# Autodesk Inventor assembly: Assembly
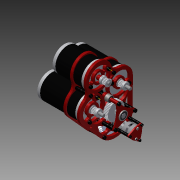
[picture p0: Inventor's stored thumbnail of the model, 180x180]
Saved by Autodesk Inventor 2013 (Build 170138000, 138)
## iProperties
Created: 2013-06-04
Part Number: Assembly
Document SubType Name: Assembly
Designer: mvarma
Author: mvarma
## Documents named in this file (59)
- C:\Users\mvarma\Desktop\GRT 2013-2014 Gearbox\Mark 3\Assembly.iam
- C:\Users\mvarma\Desktop\GRT 2013-2014 Gearbox\Mark 3\Frame Segment.ipt
- C:\Users\mvarma\Desktop\GRT 2013-2014 Gearbox\Mark 3\Plates\Cim Plate.ipt
- C:\Users\mvarma\Desktop\GRT 2013-2014 Gearbox\Mark 3\Wheel Temp.ipt
- C:\Users\mvarma\Desktop\GRT 2013-2014 Gearbox\Mark 3\Motors\Mini CIM Motor.ipt
- C:\Users\mvarma\Desktop\GRT 2013-2014 Gearbox\Mark 3\Motors\CIM Motor.ipt
- C:\Users\mvarma\Desktop\GRT 2013-2014 Gearbox\Mark 3\Pulleys\16T 3mm GT2 - 8mm Key Broach.ipt
- C:\Users\mvarma\Desktop\GRT 2013-2014 Gearbox\Mark 3\Pulleys\48T 3mm GT2 - .375 Hex Broach - Hubless.ipt
- C:\Users\mvarma\Desktop\GRT 2013-2014 Gearbox\Mark 3\Bearings\FR6-2ZZ - Hex.ipt
- C:\Users\mvarma\Desktop\GRT 2013-2014 Gearbox\Mark 3\Spacers\Shim 10 thou .500 Bore.ipt
- C:\Users\mvarma\Desktop\GRT 2013-2014 Gearbox\Mark 3\Bearings\R4-2RS.ipt
- C:\Users\mvarma\Desktop\GRT 2013-2014 Gearbox\Mark 3\Spacers\Belt Shaft Spacer 1.ipt
- C:\Users\mvarma\Desktop\GRT 2013-2014 Gearbox\Mark 3\Plates\Pnuematic Plate.ipt
- C:\Users\mvarma\Desktop\GRT 2013-2014 Gearbox\Mark 3\Spacers\Shim 10 thou .375 Bore.ipt
- C:\Users\mvarma\Desktop\GRT 2013-2014 Gearbox\Mark 3\Bearings\FR6-2RS.ipt
- C:\Users\mvarma\Desktop\GRT 2013-2014 Gearbox\Mark 3\Spacers\Belt Shaft Spacer 2.ipt
- C:\Users\mvarma\Desktop\GRT 2013-2014 Gearbox\Mark 3\Shafts\Cluster Shaft.ipt
- C:\Users\mvarma\Desktop\GRT 2013-2014 Gearbox\Mark 3\Gears\15T 20DP - .375 Hex Bore.ipt
- C:\Users\mvarma\Desktop\GRT 2013-2014 Gearbox\Mark 3\Gears\28T 20DP - .375 Hex Bore.ipt
- C:\Users\mvarma\Desktop\GRT 2013-2014 Gearbox\Mark 3\Spacers\MiniCim Spacer.ipt
- C:\Users\mvarma\Desktop\GRT 2013-2014 Gearbox\Mark 3\Spacers\Cim Spacer.ipt
- C:\Users\mvarma\Desktop\GRT 2013-2014 Gearbox\Mark 3\Plates\Mounting Plate.ipt
- C:\Users\mvarma\Desktop\GRT 2013-2014 Gearbox\Mark 3\Gears\35T 20DP - .188 Ball Shifting Bore.ipt
- C:\Users\mvarma\Desktop\GRT 2013-2014 Gearbox\Mark 3\Gears\48T 20DP - .188 Ball Shifting Bore.ipt
- C:\Users\mvarma\Desktop\GRT 2013-2014 Gearbox\Mark 3\Bearings\Thrust Bearing Washer - .6250 Bore.ipt
- C:\Users\mvarma\Desktop\GRT 2013-2014 Gearbox\Mark 3\Bearings\R10-Open.ipt
- C:\Users\mvarma\Desktop\GRT 2013-2014 Gearbox\Mark 3\Shafts\Output Shaft.ipt
- C:\Users\mvarma\Desktop\GRT 2013-2014 Gearbox\Mark 3\Pneumatic\Pneumatic Connector -Actuator Side.ipt
- C:\Users\mvarma\Desktop\GRT 2013-2014 Gearbox\Mark 3\Pneumatic\Mouning Standoff.ipt
- C:\Users\mvarma\Desktop\GRT 2013-2014 Gearbox\Mark 3\Bearings\FR8-2RS.ipt
- C:\Users\mvarma\Desktop\GRT 2013-2014 Gearbox\Mark 3\Spacers\Shim 10 thou .625 Bore.ipt
- C:\Users\mvarma\Desktop\GRT 2013-2014 Gearbox\Mark 3\Shafts\Output Shaft Insert.ipt
- C:\Users\mvarma\Desktop\GRT 2013-2014 Gearbox\Mark 3\Shafts\Ball Shifting Shaft.ipt
- C:\Users\mvarma\Desktop\GRT 2013-2014 Gearbox\Mark 3\Pneumatic\Pneumatic Connector -Shaft Side Cover.ipt
- C:\Users\mvarma\Desktop\GRT 2013-2014 Gearbox\Mark 3\Bolts\Button Head Cap Screw 4-40 Thread .125 Length.ipt
- C:\Users\mvarma\Desktop\GRT 2013-2014 Gearbox\Mark 3\Encoder\S4-120-250-N-S-B.ipt
- C:\Users\mvarma\Desktop\GRT 2013-2014 Gearbox\Mark 3\Shafts\Flexible Shaft Coupler 6208K411.ipt
- C:\Users\mvarma\Desktop\GRT 2013-2014 Gearbox\Mark 3\Encoder\Encoder Mount.ipt
- C:\Users\mvarma\Desktop\GRT 2013-2014 Gearbox\Mark 3\Bolts\Socket Head Cap Screw 6-32 Thread 1.500 Length.ipt
- C:\Users\mvarma\Desktop\GRT 2013-2014 Gearbox\Mark 3\Bearings\R3-2RS.ipt
- C:\Users\mvarma\Desktop\GRT 2013-2014 Gearbox\Mark 3\.0625 Spring Pin .2500 Long.ipt
- C:\Users\mvarma\Desktop\GRT 2013-2014 Gearbox\Mark 3\Pneumatic\FO_020_318_4F_2_03.iam
- C:\Users\mvarma\Desktop\GRT 2013-2014 Gearbox\Mark 3\Pneumatic\Mounting Plate.ipt
- C:\Users\mvarma\Desktop\GRT 2013-2014 Gearbox\Mark 3\Pem Nuts\4-40 Clinch Style Pem Nut .091 Minimum Panel Thickness.ipt
- C:\Users\mvarma\Desktop\GRT 2013-2014 Gearbox\Mark 3\Bolts\Socket Head Cap Screw 4-40 Thread 1.000 Length.ipt
- C:\Users\mvarma\Desktop\GRT 2013-2014 Gearbox\Mark 3\Bolts\Socket Head Cap Screw 6-32 Thread 2.250 Length.ipt
- C:\Users\mvarma\Desktop\GRT 2013-2014 Gearbox\Mark 3\Bolts\Socket Head Cap Screw 10-32 Thread .500 Length.ipt
- C:\Users\mvarma\Desktop\GRT 2013-2014 Gearbox\Mark 3\Spacers\Cluster Shaft Spacer.ipt
- C:\Users\mvarma\Desktop\GRT 2013-2014 Gearbox\Mark 3\Shafts\Tensioning Shaft.ipt
- C:\Users\mvarma\Desktop\GRT 2013-2014 Gearbox\Base Parts\Pulleys\22T 5mm GT2 - .500 Hex Broach.ipt
- C:\Users\mvarma\Desktop\GRT 2013-2014 Gearbox\Mark 3\Shafts\Output Shaft Hex Sleave.ipt
- C:\Users\mvarma\Desktop\GRT 2013-2014 Gearbox\Base Parts\Shafts\Base OutputShaft.ipt
- C:\Users\mvarma\Desktop\GRT 2013-2014 Gearbox\Mark 3\Bolts\Button Head Cap Screw .25-20 Thread 3.500 Length.ipt
- C:\Users\mvarma\Desktop\GRT 2013-2014 Gearbox\Mark 3\Spacers\Washer 50 thou .250 Bore.ipt
- C:\Users\mvarma\Desktop\GRT 2013-2014 Gearbox\Mark 3\Plates\Supporting Plate Standoff.ipt
- C:\Users\mvarma\Desktop\GRT 2013-2014 Gearbox\Mark 3\Plates\Main Connecting Standoff.ipt
- C:\Users\mvarma\Desktop\GRT 2013-2014 Gearbox\Mark 3\Pem Nuts\10-32 Clinch Style Pem Nut .091 Minimum Panel Thickness.ipt
- C:\Users\mvarma\Desktop\GRT 2013-2014 Gearbox\Mark 3\Bolts\Socket Head Cap Screw 10-32 Thread 3.000 Length.ipt
- C:\Users\mvarma\Desktop\GRT 2013-2014 Gearbox\Mark 3\Bolts\Socket Head Cap Screw 10-32 Thread 1.750 Length.ipt
## Components (100 placed, 57 different names)
1. Frame Segment:1 — Mate:1, Mate:2, Mate:70, Mate:71, Mate:339, Mate:340, Mate:342, Mate:343, Mate:344, Angle:6
2. Wheel Temp:1 — Mate:2, Mate:346, Mate:349
3. 22T 5mm GT2 - .500 Hex Broach:1 — Mate:339, Mate:340
4. FR8-2RS:3 — Mate:342, Mate:343, Mate:346, Mate:347
5. Output Shaft Hex Sleave:1 — Mate:344, Mate:345, Flush:26, Flush:27
6. Base OutputShaft:1 — Mate:347, Mate:348, Flush:27, Mate:349, Mate:350, Mate:352
7. Button Head Cap Screw .25-20 Thread 3.500 Length:1 — Mate:350, Mate:351, Mate:353
8. Washer 50 thou .250 Bore:1 — Mate:351, Mate:352, Mate:353
9. Supporting Plate Standoff:1 — Mate:360, Mate:361
10. Supporting Plate Standoff:2 — Mate:358, Mate:359
11. Tensioning Shaft:1 — Mate:362, Mate:363, Mate:364, Mate:365, Mate:366, Mate:367
12. Main Connecting Standoff:1 — Mate:370, Mate:371
13. Main Connecting Standoff:2 — Mate:372, Mate:373
14. Main Connecting Standoff:3 — Mate:368, Mate:369
15. 10-32 Clinch Style Pem Nut .091 Minimum Panel Thickness:1 — Mate:378, Mate:379
16. 10-32 Clinch Style Pem Nut .091 Minimum Panel Thickness:2 — Mate:376, Mate:377
17. 10-32 Clinch Style Pem Nut .091 Minimum Panel Thickness:3 — Mate:374, Mate:375
18. Socket Head Cap Screw 10-32 Thread 3.000 Length:1 — Mate:384, Mate:385
19. Socket Head Cap Screw 10-32 Thread 3.000 Length:2 — Mate:382, Mate:383
20. Socket Head Cap Screw 10-32 Thread 3.000 Length:3 — Mate:380, Mate:381
21. 10-32 Clinch Style Pem Nut .091 Minimum Panel Thickness:4 — Mate:387, Mate:388
22. 10-32 Clinch Style Pem Nut .091 Minimum Panel Thickness:5 — Mate:386, Mate:389
23. Socket Head Cap Screw 10-32 Thread 1.750 Length:1 — Mate:391, Mate:392, Mate:394
24. Socket Head Cap Screw 10-32 Thread 1.750 Length:2 — Mate:390, Mate:393, Mate:396
25. Main Connecting Standoff:4 — Mate:396, Mate:397
26. Main Connecting Standoff:5 — Mate:394, Mate:395
27. Main Connecting Standoff:6 — Mate:398, Mate:401
28. Main Connecting Standoff:7 — Mate:402, Mate:403
29. 10-32 Clinch Style Pem Nut .091 Minimum Panel Thickness:6 — Mate:404, Mate:407
30. 10-32 Clinch Style Pem Nut .091 Minimum Panel Thickness:7 — Mate:405, Mate:406
31. Socket Head Cap Screw 10-32 Thread 1.750 Length:3 — Mate:410, Mate:411
32. Socket Head Cap Screw 10-32 Thread 1.750 Length:4 — Mate:408, Mate:409
33. R10-Open:2 — Mate:218, Mate:219
34. R10-Open:1 — Mate:217, Mate:220, Mate:224
35. FR8-2RS:1 — Mate:203, Mate:204, Mate:205, Mate:208
36. FR8-2RS:2 — Mate:215, Mate:216, Mate:229, Mate:275
37. FR6-2RS:2 — Mate:74, Mate:75, Flush:24, Mate:328
38. FR6-2RS:1 — Mate:36, Mate:37, Mate:38
39. FR6-2ZZ - Hex:1 — Mate:19, Mate:20, Mate:22, Mate:44, Mate:324, Mate:325, Mate:327
40. R4-2RS:1 — Mate:27, Mate:28, Flush:9
41. R4-2RS:2 — Mate:27, Mate:28, Mate:42, Mate:364
42. Socket Head Cap Screw 6-32 Thread 1.500 Length:1 — Mate:268, Mate:270
43. Socket Head Cap Screw 6-32 Thread 1.500 Length:2 — Mate:269, Mate:271
44. S4-120-250-N-S-B:1 — Mate:263, Mate:267, Mate:272, Mate:273
45. Flexible Shaft Coupler 6208K411:1 — Mate:264, Mate:265, Mate:267
46. Encoder Mount:1 — Mate:268, Mate:269, Mate:270, Mate:271, Mate:272, Mate:273, Mate:274
47. Mounting Plate:1 — Mate:70, Mate:71, Mate:74, Mate:75, Mate:177, Mate:203, Mate:204, Mate:274, Mate:368, Mate:369, Mate:370, Mate:371, Mate:374, Mate:375, Mate:376, Mate:377, Mate:378, Mate:379, Mate:386, Mate:387, Mate:388, Mate:389, Mate:395, Mate:397, Mate:401, Mate:402, Mate:403, Mate:404, Mate:405, Mate:406, Mate:407
48. Pnuematic Plate:1 — Mate:32, Mate:34, Mate:36, Mate:37, Mate:43, Mate:367, Mate:380, Mate:381, Mate:382, Mate:383, Mate:384, Mate:385
49. Cim Plate:1 — Mate:1, Mate:3, Mate:4, Mate:5, Mate:6, Mate:7, Mate:8, Mate:9, Mate:10, Mate:11, Mate:15, Mate:19, Mate:20, Mate:21, Mate:31, Mate:32, Mate:46, Mate:215, Mate:216, Mate:288, Mate:289, Mate:292, Mate:293, Mate:294, Mate:295, Mate:312, Mate:313, Mate:314, Mate:315, Mate:316, Mate:317, Mate:318, Mate:319, Mate:320, Mate:321, Mate:322, Mate:323, Mate:358, Mate:359, Mate:360, Mate:361, Mate:362, Mate:363, Mate:372, Mate:373, Mate:390, Mate:391, Mate:392, Mate:393, Mate:398, Angle:6, Mate:408, Mate:409, Mate:410, Mate:411
50. 16T 3mm GT2 - 8mm Key Broach:1 — Mate:13, Flush:5, Flush:6
51. 16T 3mm GT2 - 8mm Key Broach:2 — Mate:12, Flush:4, Flush:7
52. 16T 3mm GT2 - 8mm Key Broach:3 — Mate:14, Flush:3, Mate:311
53. 48T 3mm GT2 - .375 Hex Broach - Hubless:1 — Mate:15, Flush:6, Flush:7, Mate:23, Flush:9, Mate:310, Mate:311, Mate:329
54. Socket Head Cap Screw 10-32 Thread .500 Length:1 — Mate:316, Mate:317
55. Socket Head Cap Screw 10-32 Thread .500 Length:2 — Mate:320, Mate:321
56. Socket Head Cap Screw 10-32 Thread .500 Length:3 — Mate:322, Mate:323
57. Socket Head Cap Screw 10-32 Thread .500 Length:4 — Mate:318, Mate:319
58. Socket Head Cap Screw 10-32 Thread .500 Length:5 — Mate:312, Mate:313
59. Socket Head Cap Screw 10-32 Thread .500 Length:6 — Mate:314, Mate:315
60. Mini CIM Motor:1 — Mate:3, Mate:4, Mate:5, Mate:14, Flush:3, Mate:51, Mate:52
61. CIM Motor:1 — Mate:9, Mate:10, Mate:11, Mate:12, Flush:4, Mate:53, Mate:54, Mate:177
62. CIM Motor:2 — Mate:6, Mate:7, Mate:8, Mate:13, Flush:5, Mate:55, Mate:56
63. Cluster Shaft Spacer:1 — Mate:327, Mate:328
64. Thrust Bearing Washer - .6250 Bore:3 — Mate:222, Mate:223, Mate:224
65. Thrust Bearing Washer - .6250 Bore:4 — Mate:225, Mate:226, Mate:228
66. Belt Shaft Spacer 1:1 — Mate:31, Mate:365
67. Belt Shaft Spacer 2:1 — Mate:42, Mate:366
68. MiniCim Spacer:1 — Mate:51, Mate:52
69. Cim Spacer:1 — Mate:53, Mate:54
70. Cim Spacer:2 — Mate:55, Mate:56
71. Shim 10 thou .500 Bore:2 — Mate:207, Mate:208, Mate:341
72. Shim 10 thou .625 Bore:2 — Mate:227, Mate:228, Mate:275
73. Shim 10 thou .375 Bore:1 — Mate:34, Mate:38, Mate:329
74. Shim 10 thou .500 Bore:1 — Mate:21, Mate:22, Mate:23
75. Output Shaft:2 — Mate:205, Mate:207, Mate:213, Mate:214, Mate:223, Mate:225, Mate:227, Mate:229, Mate:230, Mate:231, Mate:341, Mate:345, Flush:26, Mate:348
76. Cluster Shaft:1 — Mate:43, Mate:44, Angle:4, Mate:263, Mate:264, Mate:265, Mate:310, Flush:24
77. Output Shaft Insert:1 — Mate:230, Mate:231, Mate:232, Flush:23
78. Ball Shifting Shaft:1 — Mate:232, Mate:248, Flush:23, Mate:276, Mate:278, Mate:279, Mate:281
79. 35T 20DP - .188 Ball Shifting Bore:1 — Mate:213, Mate:218, Mate:219, Mate:222
80. 48T 20DP - .188 Ball Shifting Bore:1 — Mate:214, Mate:217, Mate:220, Mate:226
81. 15T 20DP - .375 Hex Bore:1 — Angle:4, Angle:5, Mate:324, Mate:325, Mate:326
82. 28T 20DP - .375 Hex Bore:1 — Mate:46, Angle:5, Mate:326
83. FO_020_318_4F_2_03:1 [sub-assembly] — Mate:282, Mate:283, Mate:284, Mate:286, Mate:287, Mate:302, Mate:303
84. 4-40 Clinch Style Pem Nut .091 Minimum Panel Thickness:1 — Mate:297, Mate:298, Mate:300
85. 4-40 Clinch Style Pem Nut .091 Minimum Panel Thickness:2 — Mate:296, Mate:299, Mate:301
86. Socket Head Cap Screw 4-40 Thread 1.000 Length:1 — Mate:301, Mate:303
87. Socket Head Cap Screw 4-40 Thread 1.000 Length:2 — Mate:300, Mate:302
88. Socket Head Cap Screw 6-32 Thread 2.250 Length:1 — Mate:304, Mate:308, Mate:338
89. Socket Head Cap Screw 6-32 Thread 2.250 Length:2 — Mate:307, Mate:400
90. Socket Head Cap Screw 6-32 Thread 2.250 Length:3 — Mate:309, Mate:399
91. Mounting Plate:2 — Mate:286, Mate:287, Mate:291, Mate:296, Mate:297, Mate:298, Mate:299, Mate:304, Mate:307, Mate:308, Mate:309
92. Mouning Standoff:1 — Mate:288, Mate:289, Mate:291, Mate:399
93. Mouning Standoff:2 — Mate:294, Mate:295, Mate:338
94. Mouning Standoff:3 — Mate:292, Mate:293, Mate:400
95. .0625 Spring Pin .2500 Long:1 — Mate:278, Mate:279
96. R3-2RS:1 — Mate:276, Mate:280, Mate:281
97. Button Head Cap Screw 4-40 Thread .125 Length:1 — Mate:259, Mate:260
98. Button Head Cap Screw 4-40 Thread .125 Length:2 — Mate:261, Mate:262
99. Pneumatic Connector -Actuator Side:1 — Mate:249, Mate:250, Mate:258, Mate:259, Mate:280, Mate:282, Mate:283, Mate:284
100. Pneumatic Connector -Shaft Side Cover:1 — Mate:248, Mate:249, Mate:250, Mate:258, Mate:260, Mate:261, Mate:262
## Relationships (219: Mate 206, Flush 10, Angle 3)
- Mate:1: Frame Segment:1 ↔ Cim Plate:1
- Mate:2: Frame Segment:1 ↔ Wheel Temp:1
- Mate:3: Cim Plate:1 ↔ Mini CIM Motor:1
- Mate:4: Cim Plate:1 ↔ Mini CIM Motor:1
- Mate:5: Cim Plate:1 ↔ Mini CIM Motor:1
- Mate:6: Cim Plate:1 ↔ CIM Motor:2
- Mate:7: Cim Plate:1 ↔ CIM Motor:2
- Mate:8: Cim Plate:1 ↔ CIM Motor:2
- Mate:9: Cim Plate:1 ↔ CIM Motor:1
- Mate:10: Cim Plate:1 ↔ CIM Motor:1
- Mate:11: Cim Plate:1 ↔ CIM Motor:1
- Mate:12: 16T 3mm GT2 - 8mm Key Broach:2 ↔ CIM Motor:1
- Mate:13: 16T 3mm GT2 - 8mm Key Broach:1 ↔ CIM Motor:2
- Mate:14: 16T 3mm GT2 - 8mm Key Broach:3 ↔ Mini CIM Motor:1
- Flush:3: 16T 3mm GT2 - 8mm Key Broach:3 ↔ Mini CIM Motor:1
- Flush:4: 16T 3mm GT2 - 8mm Key Broach:2 ↔ CIM Motor:1
- Flush:5: 16T 3mm GT2 - 8mm Key Broach:1 ↔ CIM Motor:2
- Mate:15: Cim Plate:1 ↔ 48T 3mm GT2 - .375 Hex Broach - Hubless:1
- Flush:6: 16T 3mm GT2 - 8mm Key Broach:1 ↔ 48T 3mm GT2 - .375 Hex Broach - Hubless:1
- Flush:7: 16T 3mm GT2 - 8mm Key Broach:2 ↔ 48T 3mm GT2 - .375 Hex Broach - Hubless:1
- Mate:19: FR6-2ZZ - Hex:1 ↔ Cim Plate:1
- Mate:20: FR6-2ZZ - Hex:1 ↔ Cim Plate:1
- Mate:21: Cim Plate:1 ↔ Shim 10 thou .500 Bore:1
- Mate:22: FR6-2ZZ - Hex:1 ↔ Shim 10 thou .500 Bore:1
- Mate:23: 48T 3mm GT2 - .375 Hex Broach - Hubless:1 ↔ Shim 10 thou .500 Bore:1
- Mate:27: R4-2RS:1 ↔ R4-2RS:2
- Mate:28: R4-2RS:1 ↔ R4-2RS:2
- Flush:9: R4-2RS:1 ↔ 48T 3mm GT2 - .375 Hex Broach - Hubless:1
- Mate:31: Cim Plate:1 ↔ Belt Shaft Spacer 1:1
- Mate:32: Pnuematic Plate:1 ↔ Cim Plate:1
- Mate:34: Pnuematic Plate:1 ↔ Shim 10 thou .375 Bore:1
- Mate:36: FR6-2RS:1 ↔ Pnuematic Plate:1
- Mate:37: FR6-2RS:1 ↔ Pnuematic Plate:1
- Mate:38: FR6-2RS:1 ↔ Shim 10 thou .375 Bore:1
- Mate:42: R4-2RS:2 ↔ Belt Shaft Spacer 2:1
- Mate:43: Pnuematic Plate:1 ↔ Cluster Shaft:1
- Mate:44: FR6-2ZZ - Hex:1 ↔ Cluster Shaft:1
- Mate:46: Cim Plate:1 ↔ 28T 20DP - .375 Hex Bore:1
- Angle:4 (0 deg): Cluster Shaft:1 ↔ 15T 20DP - .375 Hex Bore:1
- Angle:5 (0 deg): 15T 20DP - .375 Hex Bore:1 ↔ 28T 20DP - .375 Hex Bore:1
- Mate:51: Mini CIM Motor:1 ↔ MiniCim Spacer:1
- Mate:52: Mini CIM Motor:1 ↔ MiniCim Spacer:1
- Mate:53: CIM Motor:1 ↔ Cim Spacer:1
- Mate:54: CIM Motor:1 ↔ Cim Spacer:1
- Mate:55: CIM Motor:2 ↔ Cim Spacer:2
- Mate:56: CIM Motor:2 ↔ Cim Spacer:2
- Mate:70: Frame Segment:1 ↔ Mounting Plate:1
- Mate:71: Frame Segment:1 ↔ Mounting Plate:1
- Mate:74: FR6-2RS:2 ↔ Mounting Plate:1
- Mate:75: FR6-2RS:2 ↔ Mounting Plate:1
- Mate:177: Mounting Plate:1 ↔ CIM Motor:1
- Mate:203: FR8-2RS:1 ↔ Mounting Plate:1
- Mate:204: FR8-2RS:1 ↔ Mounting Plate:1
- Mate:205: FR8-2RS:1 ↔ Output Shaft:2
- Mate:207: Shim 10 thou .500 Bore:2 ↔ Output Shaft:2
- Mate:208: FR8-2RS:1 ↔ Shim 10 thou .500 Bore:2
- Mate:213: Output Shaft:2 ↔ 35T 20DP - .188 Ball Shifting Bore:1
- Mate:214: Output Shaft:2 ↔ 48T 20DP - .188 Ball Shifting Bore:1
- Mate:215: FR8-2RS:2 ↔ Cim Plate:1
- Mate:216: FR8-2RS:2 ↔ Cim Plate:1
- Mate:217: R10-Open:1 ↔ 48T 20DP - .188 Ball Shifting Bore:1
- Mate:218: R10-Open:2 ↔ 35T 20DP - .188 Ball Shifting Bore:1
- Mate:219: R10-Open:2 ↔ 35T 20DP - .188 Ball Shifting Bore:1
- Mate:220: R10-Open:1 ↔ 48T 20DP - .188 Ball Shifting Bore:1
- Mate:222: Thrust Bearing Washer - .6250 Bore:3 ↔ 35T 20DP - .188 Ball Shifting Bore:1
- Mate:223: Thrust Bearing Washer - .6250 Bore:3 ↔ Output Shaft:2
- Mate:224: R10-Open:1 ↔ Thrust Bearing Washer - .6250 Bore:3
- Mate:225: Thrust Bearing Washer - .6250 Bore:4 ↔ Output Shaft:2
- Mate:226: Thrust Bearing Washer - .6250 Bore:4 ↔ 48T 20DP - .188 Ball Shifting Bore:1
- Mate:227: Shim 10 thou .625 Bore:2 ↔ Output Shaft:2
- Mate:228: Thrust Bearing Washer - .6250 Bore:4 ↔ Shim 10 thou .625 Bore:2
- Mate:229: FR8-2RS:2 ↔ Output Shaft:2
- Mate:230: Output Shaft:2 ↔ Output Shaft Insert:1
- Mate:231: Output Shaft:2 ↔ Output Shaft Insert:1
- Mate:232: Output Shaft Insert:1 ↔ Ball Shifting Shaft:1
- Mate:248: Ball Shifting Shaft:1 ↔ Pneumatic Connector -Shaft Side Cover:1
- Mate:249: Pneumatic Connector -Actuator Side:1 ↔ Pneumatic Connector -Shaft Side Cover:1
- Mate:250: Pneumatic Connector -Actuator Side:1 ↔ Pneumatic Connector -Shaft Side Cover:1
- Flush:23: Output Shaft Insert:1 ↔ Ball Shifting Shaft:1
- Mate:258: Pneumatic Connector -Actuator Side:1 ↔ Pneumatic Connector -Shaft Side Cover:1
- Mate:259: Button Head Cap Screw 4-40 Thread .125 Length:1 ↔ Pneumatic Connector -Actuator Side:1
- Mate:260: Button Head Cap Screw 4-40 Thread .125 Length:1 ↔ Pneumatic Connector -Shaft Side Cover:1
- Mate:261: Button Head Cap Screw 4-40 Thread .125 Length:2 ↔ Pneumatic Connector -Shaft Side Cover:1
- Mate:262: Button Head Cap Screw 4-40 Thread .125 Length:2 ↔ Pneumatic Connector -Shaft Side Cover:1
- Mate:263: S4-120-250-N-S-B:1 ↔ Cluster Shaft:1
- Mate:264: Flexible Shaft Coupler 6208K411:1 ↔ Cluster Shaft:1
- Mate:265: Flexible Shaft Coupler 6208K411:1 ↔ Cluster Shaft:1
- Mate:267: S4-120-250-N-S-B:1 ↔ Flexible Shaft Coupler 6208K411:1
- Mate:268: Socket Head Cap Screw 6-32 Thread 1.500 Length:1 ↔ Encoder Mount:1
- Mate:269: Socket Head Cap Screw 6-32 Thread 1.500 Length:2 ↔ Encoder Mount:1
- Mate:270: Socket Head Cap Screw 6-32 Thread 1.500 Length:1 ↔ Encoder Mount:1
- Mate:271: Socket Head Cap Screw 6-32 Thread 1.500 Length:2 ↔ Encoder Mount:1
- Mate:272: S4-120-250-N-S-B:1 ↔ Encoder Mount:1
- Mate:273: S4-120-250-N-S-B:1 ↔ Encoder Mount:1
- Mate:274: Encoder Mount:1 ↔ Mounting Plate:1
- Mate:275: FR8-2RS:2 ↔ Shim 10 thou .625 Bore:2
- Mate:276: Ball Shifting Shaft:1 ↔ R3-2RS:1
- Mate:278: Ball Shifting Shaft:1 ↔ .0625 Spring Pin .2500 Long:1
- Mate:279: Ball Shifting Shaft:1 ↔ .0625 Spring Pin .2500 Long:1
- Mate:280: R3-2RS:1 ↔ Pneumatic Connector -Actuator Side:1
- Mate:281: Ball Shifting Shaft:1 ↔ R3-2RS:1
- Mate:282: FO_020_318_4F_2_03:1 ↔ Pneumatic Connector -Actuator Side:1
- Mate:283: FO_020_318_4F_2_03:1 ↔ Pneumatic Connector -Actuator Side:1
- Mate:284: FO_020_318_4F_2_03:1 ↔ Pneumatic Connector -Actuator Side:1
- Mate:286: FO_020_318_4F_2_03:1 ↔ Mounting Plate:2
- Mate:287: FO_020_318_4F_2_03:1 ↔ Mounting Plate:2
- Mate:288: Cim Plate:1 ↔ Mouning Standoff:1
- Mate:289: Cim Plate:1 ↔ Mouning Standoff:1
- Mate:291: Mounting Plate:2 ↔ Mouning Standoff:1
- Mate:292: Cim Plate:1 ↔ Mouning Standoff:3
- Mate:293: Cim Plate:1 ↔ Mouning Standoff:3
- Mate:294: Cim Plate:1 ↔ Mouning Standoff:2
- Mate:295: Cim Plate:1 ↔ Mouning Standoff:2
- Mate:296: 4-40 Clinch Style Pem Nut .091 Minimum Panel Thickness:2 ↔ Mounting Plate:2
- Mate:297: 4-40 Clinch Style Pem Nut .091 Minimum Panel Thickness:1 ↔ Mounting Plate:2
- Mate:298: 4-40 Clinch Style Pem Nut .091 Minimum Panel Thickness:1 ↔ Mounting Plate:2
- Mate:299: 4-40 Clinch Style Pem Nut .091 Minimum Panel Thickness:2 ↔ Mounting Plate:2
- Mate:300: 4-40 Clinch Style Pem Nut .091 Minimum Panel Thickness:1 ↔ Socket Head Cap Screw 4-40 Thread 1.000 Length:2
- Mate:301: 4-40 Clinch Style Pem Nut .091 Minimum Panel Thickness:2 ↔ Socket Head Cap Screw 4-40 Thread 1.000 Length:1
- Mate:302: FO_020_318_4F_2_03:1 ↔ Socket Head Cap Screw 4-40 Thread 1.000 Length:2
- Mate:303: FO_020_318_4F_2_03:1 ↔ Socket Head Cap Screw 4-40 Thread 1.000 Length:1
- Mate:304: Socket Head Cap Screw 6-32 Thread 2.250 Length:1 ↔ Mounting Plate:2
- Mate:307: Socket Head Cap Screw 6-32 Thread 2.250 Length:2 ↔ Mounting Plate:2
- Mate:308: Socket Head Cap Screw 6-32 Thread 2.250 Length:1 ↔ Mounting Plate:2
- Mate:309: Socket Head Cap Screw 6-32 Thread 2.250 Length:3 ↔ Mounting Plate:2
- Mate:310: 48T 3mm GT2 - .375 Hex Broach - Hubless:1 ↔ Cluster Shaft:1
- Mate:311: 16T 3mm GT2 - 8mm Key Broach:3 ↔ 48T 3mm GT2 - .375 Hex Broach - Hubless:1
- Mate:312: Cim Plate:1 ↔ Socket Head Cap Screw 10-32 Thread .500 Length:5
- Mate:313: Cim Plate:1 ↔ Socket Head Cap Screw 10-32 Thread .500 Length:5
- Mate:314: Cim Plate:1 ↔ Socket Head Cap Screw 10-32 Thread .500 Length:6
- Mate:315: Cim Plate:1 ↔ Socket Head Cap Screw 10-32 Thread .500 Length:6
- Mate:316: Cim Plate:1 ↔ Socket Head Cap Screw 10-32 Thread .500 Length:1
- Mate:317: Cim Plate:1 ↔ Socket Head Cap Screw 10-32 Thread .500 Length:1
- Mate:318: Cim Plate:1 ↔ Socket Head Cap Screw 10-32 Thread .500 Length:4
- Mate:319: Cim Plate:1 ↔ Socket Head Cap Screw 10-32 Thread .500 Length:4
- Mate:320: Cim Plate:1 ↔ Socket Head Cap Screw 10-32 Thread .500 Length:2
- Mate:321: Cim Plate:1 ↔ Socket Head Cap Screw 10-32 Thread .500 Length:2
- Mate:322: Cim Plate:1 ↔ Socket Head Cap Screw 10-32 Thread .500 Length:3
- Mate:323: Cim Plate:1 ↔ Socket Head Cap Screw 10-32 Thread .500 Length:3
- Mate:324: FR6-2ZZ - Hex:1 ↔ 15T 20DP - .375 Hex Bore:1
- Mate:325: FR6-2ZZ - Hex:1 ↔ 15T 20DP - .375 Hex Bore:1
- Mate:326: 15T 20DP - .375 Hex Bore:1 ↔ 28T 20DP - .375 Hex Bore:1
- Mate:327: FR6-2ZZ - Hex:1 ↔ Cluster Shaft Spacer:1
- Flush:24: FR6-2RS:2 ↔ Cluster Shaft:1
- Mate:328: FR6-2RS:2 ↔ Cluster Shaft Spacer:1
- Mate:329: 48T 3mm GT2 - .375 Hex Broach - Hubless:1 ↔ Shim 10 thou .375 Bore:1
- Mate:338: Socket Head Cap Screw 6-32 Thread 2.250 Length:1 ↔ Mouning Standoff:2
- Mate:339: Frame Segment:1 ↔ 22T 5mm GT2 - .500 Hex Broach:1
- Mate:340: Frame Segment:1 ↔ 22T 5mm GT2 - .500 Hex Broach:1
- Mate:341: Shim 10 thou .500 Bore:2 ↔ Output Shaft:2
- Mate:342: Frame Segment:1 ↔ FR8-2RS:3
- Mate:343: Frame Segment:1 ↔ FR8-2RS:3
- Mate:344: Frame Segment:1 ↔ Output Shaft Hex Sleave:1
- Mate:345: Output Shaft Hex Sleave:1 ↔ Output Shaft:2
- Flush:26: Output Shaft Hex Sleave:1 ↔ Output Shaft:2
- Mate:346: Wheel Temp:1 ↔ FR8-2RS:3
- Mate:347: FR8-2RS:3 ↔ Base OutputShaft:1
- Mate:348: Base OutputShaft:1 ↔ Output Shaft:2
- Flush:27: Output Shaft Hex Sleave:1 ↔ Base OutputShaft:1
- Mate:349: Wheel Temp:1 ↔ Base OutputShaft:1
- Mate:350: Base OutputShaft:1 ↔ Button Head Cap Screw .25-20 Thread 3.500 Length:1
- Mate:351: Button Head Cap Screw .25-20 Thread 3.500 Length:1 ↔ Washer 50 thou .250 Bore:1
- Mate:352: Base OutputShaft:1 ↔ Washer 50 thou .250 Bore:1
- Mate:353: Button Head Cap Screw .25-20 Thread 3.500 Length:1 ↔ Washer 50 thou .250 Bore:1
- Mate:358: Supporting Plate Standoff:2 ↔ Cim Plate:1
- Mate:359: Supporting Plate Standoff:2 ↔ Cim Plate:1
- Mate:360: Supporting Plate Standoff:1 ↔ Cim Plate:1
- Mate:361: Supporting Plate Standoff:1 ↔ Cim Plate:1
- Mate:362: Tensioning Shaft:1 ↔ Cim Plate:1
- Mate:363: Tensioning Shaft:1 ↔ Cim Plate:1
- Mate:364: Tensioning Shaft:1 ↔ R4-2RS:2
- Mate:365: Tensioning Shaft:1 ↔ Belt Shaft Spacer 1:1
- Mate:366: Tensioning Shaft:1 ↔ Belt Shaft Spacer 2:1
- Mate:367: Tensioning Shaft:1 ↔ Pnuematic Plate:1
- Mate:368: Main Connecting Standoff:3 ↔ Mounting Plate:1
- Mate:369: Main Connecting Standoff:3 ↔ Mounting Plate:1
- Mate:370: Main Connecting Standoff:1 ↔ Mounting Plate:1
- Mate:371: Main Connecting Standoff:1 ↔ Mounting Plate:1
- Mate:372: Main Connecting Standoff:2 ↔ Cim Plate:1
- Mate:373: Main Connecting Standoff:2 ↔ Cim Plate:1
- Mate:374: 10-32 Clinch Style Pem Nut .091 Minimum Panel Thickness:3 ↔ Mounting Plate:1
- Mate:375: 10-32 Clinch Style Pem Nut .091 Minimum Panel Thickness:3 ↔ Mounting Plate:1
- Mate:376: 10-32 Clinch Style Pem Nut .091 Minimum Panel Thickness:2 ↔ Mounting Plate:1
- Mate:377: 10-32 Clinch Style Pem Nut .091 Minimum Panel Thickness:2 ↔ Mounting Plate:1
- Mate:378: 10-32 Clinch Style Pem Nut .091 Minimum Panel Thickness:1 ↔ Mounting Plate:1
- Mate:379: 10-32 Clinch Style Pem Nut .091 Minimum Panel Thickness:1 ↔ Mounting Plate:1
- Mate:380: Socket Head Cap Screw 10-32 Thread 3.000 Length:3 ↔ Pnuematic Plate:1
- Mate:381: Socket Head Cap Screw 10-32 Thread 3.000 Length:3 ↔ Pnuematic Plate:1
- Mate:382: Socket Head Cap Screw 10-32 Thread 3.000 Length:2 ↔ Pnuematic Plate:1
- Mate:383: Socket Head Cap Screw 10-32 Thread 3.000 Length:2 ↔ Pnuematic Plate:1
- Mate:384: Socket Head Cap Screw 10-32 Thread 3.000 Length:1 ↔ Pnuematic Plate:1
- Mate:385: Socket Head Cap Screw 10-32 Thread 3.000 Length:1 ↔ Pnuematic Plate:1
- Mate:386: 10-32 Clinch Style Pem Nut .091 Minimum Panel Thickness:5 ↔ Mounting Plate:1
- Mate:387: 10-32 Clinch Style Pem Nut .091 Minimum Panel Thickness:4 ↔ Mounting Plate:1
- Mate:388: 10-32 Clinch Style Pem Nut .091 Minimum Panel Thickness:4 ↔ Mounting Plate:1
- Mate:389: 10-32 Clinch Style Pem Nut .091 Minimum Panel Thickness:5 ↔ Mounting Plate:1
- Mate:390: Socket Head Cap Screw 10-32 Thread 1.750 Length:2 ↔ Cim Plate:1
- Mate:391: Socket Head Cap Screw 10-32 Thread 1.750 Length:1 ↔ Cim Plate:1
- Mate:392: Socket Head Cap Screw 10-32 Thread 1.750 Length:1 ↔ Cim Plate:1
- Mate:393: Socket Head Cap Screw 10-32 Thread 1.750 Length:2 ↔ Cim Plate:1
- Mate:394: Socket Head Cap Screw 10-32 Thread 1.750 Length:1 ↔ Main Connecting Standoff:5
- Mate:395: Main Connecting Standoff:5 ↔ Mounting Plate:1
- Mate:396: Socket Head Cap Screw 10-32 Thread 1.750 Length:2 ↔ Main Connecting Standoff:4
- Mate:397: Main Connecting Standoff:4 ↔ Mounting Plate:1
- Mate:398: Main Connecting Standoff:6 ↔ Cim Plate:1
- Mate:399: Socket Head Cap Screw 6-32 Thread 2.250 Length:3 ↔ Mouning Standoff:1
- Mate:400: Socket Head Cap Screw 6-32 Thread 2.250 Length:2 ↔ Mouning Standoff:3
- Angle:6 (180 deg): Frame Segment:1 ↔ Cim Plate:1
- Mate:401: Main Connecting Standoff:6 ↔ Mounting Plate:1
- Mate:402: Main Connecting Standoff:7 ↔ Mounting Plate:1
- Mate:403: Main Connecting Standoff:7 ↔ Mounting Plate:1
- Mate:404: 10-32 Clinch Style Pem Nut .091 Minimum Panel Thickness:6 ↔ Mounting Plate:1
- Mate:405: 10-32 Clinch Style Pem Nut .091 Minimum Panel Thickness:7 ↔ Mounting Plate:1
- Mate:406: 10-32 Clinch Style Pem Nut .091 Minimum Panel Thickness:7 ↔ Mounting Plate:1
- Mate:407: 10-32 Clinch Style Pem Nut .091 Minimum Panel Thickness:6 ↔ Mounting Plate:1
- Mate:408: Socket Head Cap Screw 10-32 Thread 1.750 Length:4 ↔ Cim Plate:1
- Mate:409: Socket Head Cap Screw 10-32 Thread 1.750 Length:4 ↔ Cim Plate:1
- Mate:410: Socket Head Cap Screw 10-32 Thread 1.750 Length:3 ↔ Cim Plate:1
- Mate:411: Socket Head Cap Screw 10-32 Thread 1.750 Length:3 ↔ Cim Plate:1
